# Autodesk Inventor assembly: main
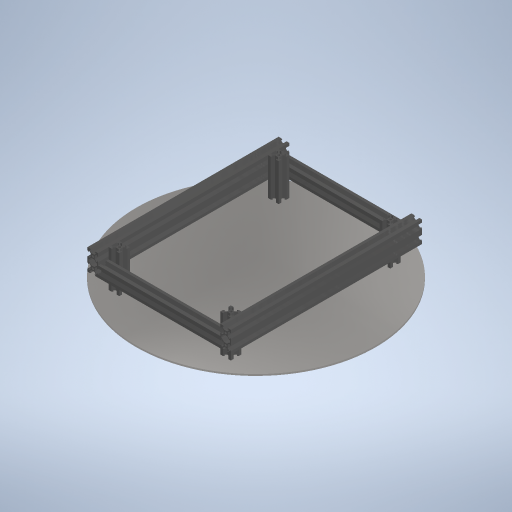
[picture p0: Inventor's stored thumbnail of the model, 512x512]
Saved by Autodesk Inventor 2024.2 (Build 282272000, 272)
## iProperties
Created: 2024-08-26
Part Number: main
Document SubType Name: Assembly
Designer: Admin
Author: Admin
## Documents named in this file (3)
- C:\Users\Admin\Documents\GitHub\RobotCartesiano\DiseñoBrazo\Assemblies\main.iam
- C:\Users\Admin\Documents\GitHub\RobotCartesiano\DiseñoBrazo\Assemblies\AxisX.iam
- C:\Users\Admin\Documents\GitHub\RobotCartesiano\DiseñoBrazo\FestinoRobot\AluminumBase.ipt
## Components (2 placed, 2 different names)
1. AluminumBase:1 — Mate:1
2. AxisX:1 [sub-assembly] — Mate:1
## Relationships (1: Mate 1)
- Mate:1: AluminumBase:1 ↔ AxisX:1
